# Autodesk Inventor assembly: Cockpit_battery_frame
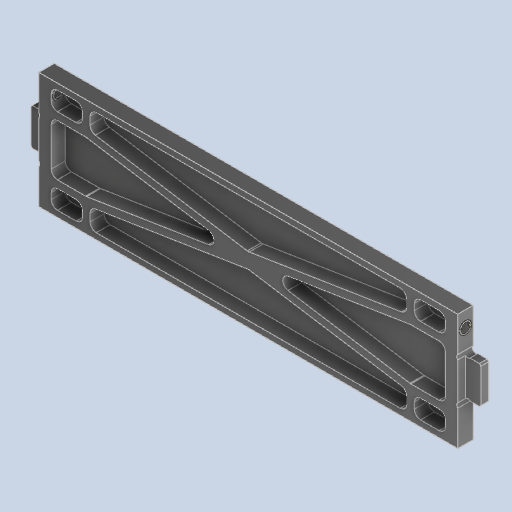
[picture p0: Inventor's stored thumbnail of the model, 512x512]
Saved by Autodesk Inventor 2022.5 (Build 265521000, 521)
## iProperties
Created: 2023-05-18
Part Number: Cockpit_battery_frame
Document SubType Name: Assembly
Designer: Masato Kubotera
Author: Masato Kubotera
## Documents named in this file (3)
- C:\Users\Masato\Documents\Inventor\SUSTAINA-OP\ModelingFiles\UpperBody\Cockpit\Cockpit_battery_frame.iam
- C:\Users\Masato\Documents\Inventor\SUSTAINA-OP\ModelingFiles\UpperBody\Cockpit\Cockpit_battery_frame.ipt
- C:\Users\Masato\Documents\Inventor\SUSTAINA-OP\ModelingFiles\COTS\InsertNut\IRU-304S.ipt
## Components (3 placed, 2 different names)
1. Cockpit_battery_frame:1 — フラッシュ:1, フラッシュ:2, フラッシュ:3, 挿入:1, 挿入:2
2. IRU-304S:1 — 挿入:1
3. IRU-304S:2 — 挿入:2
## Relationships (5: Flush 3, Insert 2)
- フラッシュ:1 [Flush]: Cockpit_battery_frame:1
- フラッシュ:2 [Flush]: Cockpit_battery_frame:1
- フラッシュ:3 [Flush]: Cockpit_battery_frame:1
- 挿入:1 [Insert]: Cockpit_battery_frame:1 ↔ IRU-304S:1
- 挿入:2 [Insert]: Cockpit_battery_frame:1 ↔ IRU-304S:2
